# Autodesk Inventor assembly: CAST
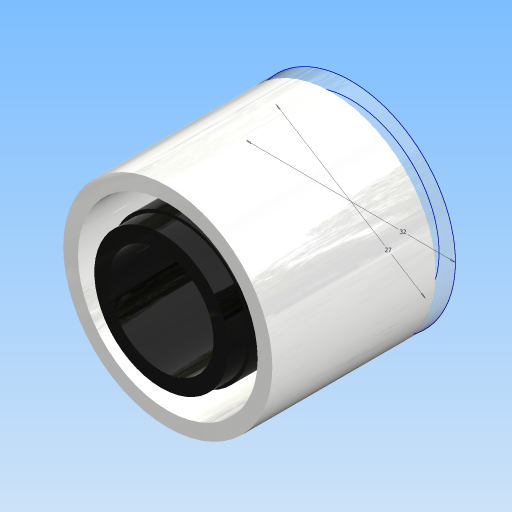
[picture p0: Inventor's stored thumbnail of the model, 512x512]
Saved by Autodesk Inventor 2024.2 (Build 282272000, 272)
## iProperties
Created: 2024-03-12
Part Number: CAST
Document SubType Name: Assembly
Designer: MenMe
Author: MenMe
## Documents named in this file (4)
- C:\Users\MenMe\GitHub\RoboCop\- 3D -\mech._parts\CAST.iam
- C:\Users\MenMe\Downloads\tyreform_bottom1.ipt
- C:\Users\MenMe\Downloads\tyreform_center1.ipt
- C:\Users\MenMe\Downloads\tyreform_sleeve1.ipt
## Components (3 placed, 3 different names)
1. tyreform_bottom1:1 — Insert:2, Insert:3
2. tyreform_center1:1 — Insert:3
3. tyreform_sleeve1:1 — Insert:2
## Relationships (2: Insert 2)
- Insert:2: tyreform_bottom1:1 ↔ tyreform_sleeve1:1
- Insert:3: tyreform_bottom1:1 ↔ tyreform_center1:1
